# Autodesk Inventor assembly: Camera_Assem
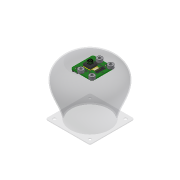
[picture p0: Inventor's stored thumbnail of the model, 180x180]
Saved by Autodesk Inventor 2018 (Build 220112000, 112)
## iProperties
Created: 2019-11-21
Part Number: Camera_Assem
Document SubType Name: Assembly
Designer: Clevo
Author: Clevo
## Documents named in this file (4)
- E:\RobotArm\MCAD\Camera_Assem.iam
- E:\RobotArm\MCAD\raspberry-pi-camera-module-v2-1.snapshot.3\RspCameraMia.iam
- E:\RobotArm\MCAD\Light_Camera.ipt
- E:\Hardware_Accelerated_Robot\Hardware\MCAD\Computers\Jetson_Standoff.ipt
## Components (6 placed, 3 different names)
1. RspCameraMia:1 [sub-assembly] — Mate:1, Mate:2, Mate:3, Mate:4, Mate:5, Mate:6, Mate:7, Mate:8
2. Light_Camera:1 — Mate:9, Mate:10, Mate:11
3. Jetson_Standoff:1 — Mate:1, Mate:4
4. Jetson_Standoff:2 — Mate:6, Mate:7
5. Jetson_Standoff:3 — Mate:5, Mate:8, Mate:10, Mate:11
6. Jetson_Standoff:4 — Mate:2, Mate:3, Mate:9
## Relationships (11: Mate 11)
- Mate:1: RspCameraMia:1 ↔ Jetson_Standoff:1
- Mate:2: RspCameraMia:1 ↔ Jetson_Standoff:4
- Mate:3: RspCameraMia:1 ↔ Jetson_Standoff:4
- Mate:4: RspCameraMia:1 ↔ Jetson_Standoff:1
- Mate:5: RspCameraMia:1 ↔ Jetson_Standoff:3
- Mate:6: RspCameraMia:1 ↔ Jetson_Standoff:2
- Mate:7: RspCameraMia:1 ↔ Jetson_Standoff:2
- Mate:8: RspCameraMia:1 ↔ Jetson_Standoff:3
- Mate:9: Light_Camera:1 ↔ Jetson_Standoff:4
- Mate:10: Light_Camera:1 ↔ Jetson_Standoff:3
- Mate:11: Light_Camera:1 ↔ Jetson_Standoff:3
